# Autodesk Inventor assembly: Full chassis 2
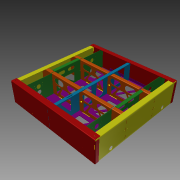
[picture p0: Inventor's stored thumbnail of the model, 180x180]
Saved by Autodesk Inventor 2015 SP1 (Build 190203100, 203)
## iProperties
Created: 2014-01-06
Part Number: Full chassis 2
Document SubType Name: Weldment
Designer: Alex
Weld Material: Welded Aluminum-6061
Mass: 8202.81 g
Surface Area: 27357.1 cm^2
Volume: 3031.7 cm^3
Density: 2.70568 g/cm^3
Author: Alex
## Documents named in this file (9)
- X:\2015 V2 A\Full chassis-3.iam
- X:\2015 V2 A\Front-3.ipt
- X:\2015 V2 A\Brace-3.ipt
- X:\2015 V2 A\InnerSide-3.ipt
- X:\2015 V2 A\Outer_Side-3.ipt
- X:\2015 V2 A\Base-3.ipt
- X:\2015 V2 A\CenterBrace-3.ipt
- X:\2015 V2 A\CenterBrace-3d.ipt
- X:\2015 V2 A\InnerSide-3-Right.ipt
## Components (11 placed, 8 different names)
1. Brace-3:1 — Mate:25, Mate:37, Mate:38, Mate:39, Mate:42, Flush:7, Mate:56, Mate:57
2. Brace-3:2 — Mate:9, Mate:24, Mate:59, Mate:60, Flush:8, Mate:61
3. Front-3:1 — Mate:9, Flush:4, Mate:41, Mate:58
4. InnerSide-3:3 — Mate:24, Mate:25, Mate:35, Mate:58
5. Front-3:2 — Mate:35, Flush:5, Mate:62
6. Base-3:1 — Mate:37, Mate:38, Mate:39, Mate:40, Flush:6, Mate:63
7. CenterBrace-3:1 — Mate:40, Flush:4, Mate:41
8. CenterBrace-3d:1 — Flush:5, Flush:6, Mate:42
9. Outer_Side-3:2 — Flush:7, Mate:56, Mate:57
10. Outer_Side-3:3 — Mate:59, Mate:60, Flush:8
11. InnerSide-3-Right:1 — Mate:61, Mate:62, Mate:63
## Relationships (23: Mate 18, Flush 5)
- Mate:9 (-228.6 mm): Brace-3:2 ↔ Front-3:1
- Mate:24: Brace-3:2 ↔ InnerSide-3:3
- Mate:25: Brace-3:1 ↔ InnerSide-3:3
- Mate:35: InnerSide-3:3 ↔ Front-3:2
- Mate:37: Brace-3:1 ↔ Base-3:1
- Mate:38: Brace-3:1 ↔ Base-3:1
- Mate:39: Brace-3:1 ↔ Base-3:1
- Mate:40: Base-3:1 ↔ CenterBrace-3:1
- Flush:4: Front-3:1 ↔ CenterBrace-3:1
- Mate:41: Front-3:1 ↔ CenterBrace-3:1
- Flush:5: Front-3:2 ↔ CenterBrace-3d:1
- Flush:6: Base-3:1 ↔ CenterBrace-3d:1
- Mate:42: Brace-3:1 ↔ CenterBrace-3d:1
- Flush:7: Brace-3:1 ↔ Outer_Side-3:2
- Mate:56: Brace-3:1 ↔ Outer_Side-3:2
- Mate:57: Brace-3:1 ↔ Outer_Side-3:2
- Mate:58: Front-3:1 ↔ InnerSide-3:3
- Mate:59: Brace-3:2 ↔ Outer_Side-3:3
- Mate:60: Brace-3:2 ↔ Outer_Side-3:3
- Flush:8: Brace-3:2 ↔ Outer_Side-3:3
- Mate:61: Brace-3:2 ↔ InnerSide-3-Right:1
- Mate:62: Front-3:2 ↔ InnerSide-3-Right:1
- Mate:63: Base-3:1 ↔ InnerSide-3-Right:1
